# Autodesk Inventor assembly: openmv3
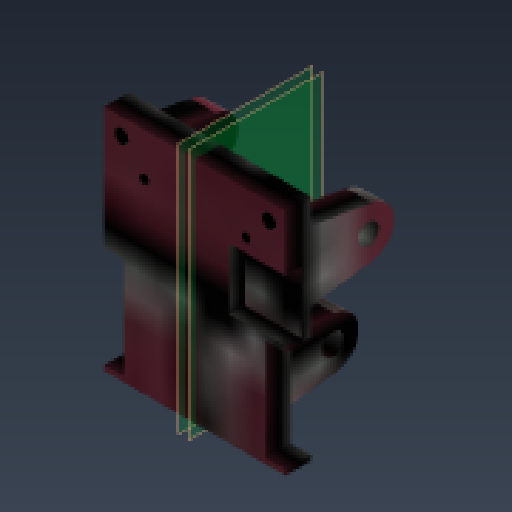
[picture p0: Inventor's stored thumbnail of the model, 512x512]
Saved by Autodesk Inventor 2023.2 (Build 272271030, 271C)
## iProperties
Created: 2018-03-12
Part Number: openmv3
Description: STEP AP214
Document SubType Name: Assembly
Designer: liza
Sending System: SolidWorks 2016
Preprocessor: SwSTEP 2.0
Title: openmv3.STEP
Revision Number: ANY
## Documents named in this file (23)
- D:\!project\fox_n_crow_construction\crow\trunk\камера+качалка.iam
- C:\Users\liza\Desktop\Work\openmv3_export\openmv3.ipt
- C:\Users\liza\Desktop\Work\openmv3_export\Capacitor 0805.ipt
- C:\Users\liza\Desktop\Work\openmv3_export\Capacitor 0603.ipt
- C:\Users\liza\Desktop\Work\openmv3_export\SOT 23.ipt
- C:\Users\liza\Desktop\Work\openmv3_export\Header 2_54 Vertical 1x5.ipt
- C:\Users\liza\Desktop\Work\openmv3_export\LED SMD RGB.ipt
- C:\Users\liza\Desktop\Work\openmv3_export\LED 1206 IR.ipt
- C:\Users\liza\Desktop\Work\openmv3_export\mount_lens.ipt
- C:\Users\liza\Desktop\Work\openmv3_export\Resistor 0603.ipt
- C:\Users\liza\Desktop\Work\openmv3_export\EXBV8V.ipt
- C:\Users\liza\Desktop\Work\openmv3_export\EXBV4V.ipt
- C:\Users\liza\Desktop\Work\openmv3_export\User Library-LQFP100-3.iam
- C:\Users\liza\Desktop\Work\openmv3_export\CSP2-28.ipt
- C:\Users\liza\Desktop\Work\openmv3_export\User Library-HSOP8_® ã¬®«ç ­¨î.iam
- C:\Users\liza\Desktop\Work\openmv3_export\uSD_socket.ipt
- C:\Users\liza\Desktop\Work\openmv3_export\UJ2-MIBH2-4-SMT_Defaut.iam
- C:\Users\liza\Desktop\Work\openmv3_export\Crystal-SM2520-4.ipt
- C:\Users\liza\Desktop\Work\openmv3_export\Capacitor 3216.ipt
- C:\Users\liza\Desktop\Work\openmv3_export\960240-6202-AR 1x8 long.iam
- C:\Users\liza\Desktop\Work\openmv3_export\pan head cross recess screw_iso_ISO 7045 - M1 x 4 - Z - 4S.ipt
- D:\!project\fox_n_crow_construction\crow\trunk\Качель камеры.ipt
- C:\Users\liza\Desktop\Work\openmv3_export\Lens\LENS_Standard.ipt
## Components (52 placed, 52 different names)
1. openmv3_1 — Совмещение:1, Заподлицо:1, Заподлицо:2
2. Capacitor 0805_2
3. Capacitor 0805_3
4. Capacitor 0805_4
5. Capacitor 0603_5
6. Capacitor 0603_6
7. Capacitor 0603_7
8. Capacitor 0603_8
9. Capacitor 0603_9
10. Capacitor 0603_10
11. Capacitor 0603_11
12. Capacitor 0603_12
13. Capacitor 0603_13
14. Capacitor 0603_14
15. Capacitor 0603_15
16. Capacitor 0603_16
17. Capacitor 0603_17
18. Capacitor 0603_18
19. Capacitor 0603_19
20. Capacitor 0603_20
21. Capacitor 0603_21
22. SOT 23_22
23. Header 2_54 Vertical 1x5_23
24. Capacitor 0603_24
25. Capacitor 0603_25
26. LED SMD RGB_26
27. LED 1206 IR_27
28. LED 1206 IR_28
29. mount_lens_29 — Совмещение:2, Совмещение:3
30. SOT 23_30
31. Resistor 0603_31
32. Resistor 0603_32
33. Resistor 0603_33
34. Resistor 0603_34
35. EXBV8V_35
36. EXBV8V_36
37. EXBV8V_37
38. EXBV4V_38
39. User Library-LQFP100-3_39 [sub-assembly]
40. CSP2-28_40
41. User Library-HSOP8_® ã¬®«ç ­¨î_41 [sub-assembly]
42. uSD_socket_42
43. UJ2-MIBH2-4-SMT_Defaut_43 [sub-assembly]
44. Crystal-SM2520-4_44
45. Capacitor 3216_45
46. Capacitor 3216_46
47. Capacitor 3216_47
48. 960240-6202-AR 1x8 long_48 [sub-assembly]
49. 960240-6202-AR 1x8 long_49 [sub-assembly]
50. pan head cross recess screw_iso_ISO 7045 - M1 x 4 - Z - 4S_50
51. Качель камеры:1 — Совмещение:1, Заподлицо:1, Заподлицо:2
52. LENS_Standard:1 — Совмещение:2, Совмещение:3
## Relationships (5: Mate 3, Flush 2)
- Совмещение:1 [Mate]: openmv3_1 ↔ Качель камеры:1
- Заподлицо:1 [Flush]: openmv3_1 ↔ Качель камеры:1
- Заподлицо:2 [Flush]: openmv3_1 ↔ Качель камеры:1
- Совмещение:2 [Mate]: mount_lens_29 ↔ LENS_Standard:1
- Совмещение:3 [Mate] (6 mm): mount_lens_29 ↔ LENS_Standard:1
